# Autodesk Inventor assembly: wall
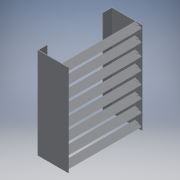
[picture p0: Inventor's stored thumbnail of the model, 180x180]
Saved by Autodesk Inventor 2019.3 (Build 233278000, 278)
## iProperties
Created: 2019-04-01
Part Number: wall
Document SubType Name: Assembly
Designer: erwin
Author: erwin
## Documents named in this file (3)
- D:\GitHub\DrowningWarnings\wave_simulator\wall\NEW_DESIGN\wall.iam
- D:\GitHub\DrowningWarnings\wave_simulator\wall\NEW_DESIGN\base.ipt
- D:\GitHub\DrowningWarnings\wave_simulator\wall\NEW_DESIGN\top.ipt
## Components (2 placed, 2 different names)
1. base:1 — Flush:1
2. top:1 — Flush:1
## Relationships (1: Flush 1)
- Flush:1: base:1 ↔ top:1
